# Autodesk Inventor assembly: Assembly_Opentrons_Imagingunit_v0
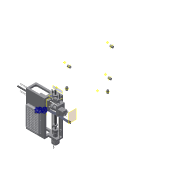
[picture p0: Inventor's stored thumbnail of the model, 180x180]
Saved by Autodesk Inventor 2019.4 (Build 234330000, 330)
## iProperties
Created: 2020-10-27
Part Number: Assembly_Opentrons_Imagingunit_v0
Document SubType Name: Assembly
Designer: diederichbenedict
Author: diederichbenedict
## Documents named in this file (8)
- C:\Users\diederichbenedict\Dropbox\Dokumente\Promotion\PROJECTS\OPENTRONS\INVENTOR\Assembly_Opentrons_Imagingunit_v0.iam
- C:\Users\diederichbenedict\Dropbox\Dokumente\Promotion\PROJECTS\OPENTRONS\INVENTOR\Assembly_Opentrons_Autofocus_v0.iam
- C:\Users\diederichbenedict\Dropbox\Dokumente\Promotion\PROJECTS\OPENTRONS\INVENTOR\00_MTP_96-welplate.ipt
- C:\Users\diederichbenedict\Dropbox\Dokumente\Promotion\PROJECTS\OPENTRONS\INVENTOR\00_IGUS_Drylin_RJ4JP-01-06.ipt
- C:\Users\diederichbenedict\Dropbox\Dokumente\Promotion\PROJECTS\OPENTRONS\INVENTOR\04_OPENTRONS_Microscope_wellplate_base.ipt
- C:\Users\diederichbenedict\Dropbox\Dokumente\Promotion\PROJECTS\OPENTRONS\INVENTOR\Assembly_opentrons_microscope_slide_y.iam
- C:\Users\diederichbenedict\Dropbox\Dokumente\Promotion\PROJECTS\OPENTRONS\INVENTOR\Assembly_opentrons_microscope_slide_y_base.iam
- C:\Users\diederichbenedict\Dropbox\Dokumente\Promotion\PROJECTS\OPENTRONS\INVENTOR\00_Endstop.ipt
## Components (11 placed, 7 different names)
1. 00_IGUS_Drylin_RJ4JP-01-06:5
2. 00_IGUS_Drylin_RJ4JP-01-06:6
3. 00_IGUS_Drylin_RJ4JP-01-06:7
4. 00_IGUS_Drylin_RJ4JP-01-06:8
5. 00_IGUS_Drylin_RJ4JP-01-06:9
6. 04_OPENTRONS_Microscope_wellplate_base:1 — Mate:8, Mate:9, Mate:10, Insert:1
7. Assembly_Opentrons_Autofocus_v0:1 [sub-assembly] — Mate:3, Mate:4
8. Assembly_opentrons_microscope_slide_y:1 [sub-assembly] — Mate:1, Mate:2, Mate:3, Mate:4, Mate:12
9. Assembly_opentrons_microscope_slide_y_base:1 [sub-assembly] — Mate:1, Flush:7, Flush:8, Flush:9, Mate:2, Mate:6, Mate:7, Mate:11, Insert:1, Angle:1, Flush:10
10. 00_MTP_96-welplate:1 — Mate:6, Mate:7, Mate:8, Mate:9, Mate:10
11. 00_Endstop:1 — Mate:11, Mate:12, Angle:1, Flush:10
## Relationships (17: Mate 11, Flush 4, Insert 1, Angle 1)
- Mate:1: Assembly_opentrons_microscope_slide_y:1 ↔ Assembly_opentrons_microscope_slide_y_base:1
- Flush:7: Assembly_opentrons_microscope_slide_y_base:1
- Flush:8: Assembly_opentrons_microscope_slide_y_base:1
- Flush:9: Assembly_opentrons_microscope_slide_y_base:1
- Mate:2: Assembly_opentrons_microscope_slide_y:1 ↔ Assembly_opentrons_microscope_slide_y_base:1
- Mate:3: Assembly_Opentrons_Autofocus_v0:1 ↔ Assembly_opentrons_microscope_slide_y:1
- Mate:4: Assembly_Opentrons_Autofocus_v0:1 ↔ Assembly_opentrons_microscope_slide_y:1
- Mate:6 (8 mm): Assembly_opentrons_microscope_slide_y_base:1 ↔ 00_MTP_96-welplate:1
- Mate:7 (18 mm): Assembly_opentrons_microscope_slide_y_base:1 ↔ 00_MTP_96-welplate:1
- Mate:8: 04_OPENTRONS_Microscope_wellplate_base:1 ↔ 00_MTP_96-welplate:1
- Mate:9 (-2 mm): 04_OPENTRONS_Microscope_wellplate_base:1 ↔ 00_MTP_96-welplate:1
- Mate:10 (-2 mm): 04_OPENTRONS_Microscope_wellplate_base:1 ↔ 00_MTP_96-welplate:1
- Mate:11: Assembly_opentrons_microscope_slide_y_base:1 ↔ 00_Endstop:1
- Insert:1: 04_OPENTRONS_Microscope_wellplate_base:1 ↔ Assembly_opentrons_microscope_slide_y_base:1
- Mate:12: Assembly_opentrons_microscope_slide_y:1 ↔ 00_Endstop:1
- Angle:1 (180 deg): Assembly_opentrons_microscope_slide_y_base:1 ↔ 00_Endstop:1
- Flush:10 (10 mm): Assembly_opentrons_microscope_slide_y_base:1 ↔ 00_Endstop:1
